# Autodesk Inventor assembly: Shaft
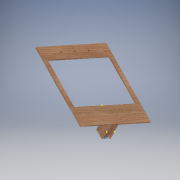
[picture p0: Inventor's stored thumbnail of the model, 180x180]
Saved by Autodesk Inventor 2016 (Build 200138000, 138)
## iProperties
Created: 2016-05-06
Part Number: Shaft
Document SubType Name: Assembly
Designer: mkepler
Author: mkepler
## Documents named in this file (5)
- C:\Users\mkepler\Google Drive\Michael Kepler\College\ECE\ECE 590\Project 3\Physical Design\Inventor Files\Shaft\Shaft.iam
- C:\Users\mkepler\Google Drive\Michael Kepler\College\ECE\ECE 590\Project 3\Physical Design\Inventor Files\Shaft\Base.ipt
- C:\Users\mkepler\Google Drive\Michael Kepler\College\ECE\ECE 590\Project 3\Physical Design\Inventor Files\xl320Servo.ipt
- C:\Users\mkepler\Google Drive\Michael Kepler\College\ECE\ECE 590\Project 3\Physical Design\Inventor Files\Shaft\SideSupport.ipt
- C:\Users\mkepler\Google Drive\Michael Kepler\College\ECE\ECE 590\Project 3\Physical Design\Inventor Files\Shaft\FrontSupport.ipt
## Components (5 placed, 4 different names)
1. Base:1 — Insert:1, Insert:2, Insert:3, Insert:4, Insert:5, Insert:6, Insert:7
2. xl320Servo:1 — Insert:1, Insert:2
3. SideSupport:2 — Insert:5, Insert:6
4. FrontSupport:1 — Insert:3, Insert:4
5. SideSupport:3 — Insert:7
## Relationships (7: Insert 7)
- Insert:1: Base:1 ↔ xl320Servo:1
- Insert:2: Base:1 ↔ xl320Servo:1
- Insert:3: Base:1 ↔ FrontSupport:1
- Insert:4: Base:1 ↔ FrontSupport:1
- Insert:5: Base:1 ↔ SideSupport:2
- Insert:6: Base:1 ↔ SideSupport:2
- Insert:7: Base:1 ↔ SideSupport:3
